# Autodesk Inventor assembly: flipper lift
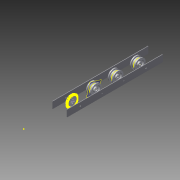
[picture p0: Inventor's stored thumbnail of the model, 180x180]
Saved by Autodesk Inventor 2015 (Build 190159000, 159)
## iProperties
Created: 2014-11-02
Part Number: flipper lift
Document SubType Name: Assembly
Designer: jesse
Author: jesse
## Documents named in this file (6)
- C:\Users\jesse\Desktop\robot\flipper lift\flipper lift.iam
- C:\Users\jesse\Desktop\robot\flipper lift\side.ipt
- C:\Users\jesse\Desktop\robot\stock parts\tetrix_736468_tt_sprocket_2012\tetrix_736468_tt_sprocket_2012.ipt
- C:\Users\jesse\Desktop\robot\stock parts\tetrix_736468_tt_wheel_2012\tetrix_736468_tt_wheel_2012.ipt
- C:\Users\jesse\Desktop\robot\flipper lift\chain.ipt
- C:\Users\jesse\Desktop\robot\flipper lift\chain2.ipt
## Components (8 placed, 5 different names)
1. side:1 — Flush:1, Flush:2, Mate:1, Mate:2, Mate:3, Mate:4
2. side:2 — Flush:1, Flush:2
3. tetrix_736468_tt_sprocket_2012:1 — Mate:4, Flush:3
4. tetrix_736468_tt_wheel_2012:1 — Mate:3, Flush:3, Flush:4, Flush:6, Flush:8, Flush:9
5. tetrix_736468_tt_wheel_2012:2 — Mate:2, Flush:4, Flush:5
6. tetrix_736468_tt_wheel_2012:3 — Mate:1, Flush:5
7. chain:1 — Flush:7
8. chain2:1 — Flush:8, Flush:9
## Relationships (13: Flush 9, Mate 4)
- Flush:1: side:1 ↔ side:2
- Flush:2: side:1 ↔ side:2
- Mate:1: side:1 ↔ tetrix_736468_tt_wheel_2012:3
- Mate:2: side:1 ↔ tetrix_736468_tt_wheel_2012:2
- Mate:3: side:1 ↔ tetrix_736468_tt_wheel_2012:1
- Mate:4: side:1 ↔ tetrix_736468_tt_sprocket_2012:1
- Flush:3: tetrix_736468_tt_sprocket_2012:1 ↔ tetrix_736468_tt_wheel_2012:1
- Flush:4: tetrix_736468_tt_wheel_2012:1 ↔ tetrix_736468_tt_wheel_2012:2
- Flush:5: tetrix_736468_tt_wheel_2012:2 ↔ tetrix_736468_tt_wheel_2012:3
- Flush:6: tetrix_736468_tt_wheel_2012:1
- Flush:7: chain:1
- Flush:8: tetrix_736468_tt_wheel_2012:1 ↔ chain2:1
- Flush:9: tetrix_736468_tt_wheel_2012:1 ↔ chain2:1
